# Autodesk Inventor assembly: Kopula+plus_OLED
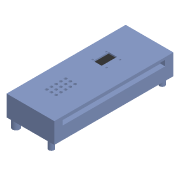
[picture p0: Inventor's stored thumbnail of the model, 180x180]
Saved by Autodesk Inventor 2021 (Build 250183000, 183)
## iProperties
Created: 2022-11-02
Part Number: Kopula+plus_OLED
Document SubType Name: Assembly
Designer: agnpi
Author: agnpi
## Documents named in this file (3)
- D:\users\agnpi\Desktop\lekcje\SEMESTR VII\INVENTOR INZ SPRAWDZONE\Kopula+plus_OLED.iam
- D:\users\agnpi\Desktop\lekcje\SEMESTR VII\INVENTOR INZ SPRAWDZONE\kopula_pod_OLED.ipt
- D:\users\agnpi\Desktop\lekcje\SEMESTR VII\INVENTOR INZ SPRAWDZONE\Pantalla OLED 0.96'' 128x64.iam
## Components (2 placed, 2 different names)
1. kopula_pod_OLED:1 — Mate:1, Mate:2, Mate:3
2. Pantalla OLED 0.96'' 128x64:1 [sub-assembly] — Mate:1, Mate:2, Mate:3
## Relationships (3: Mate 3)
- Mate:1: kopula_pod_OLED:1 ↔ Pantalla OLED 0.96'' 128x64:1
- Mate:2: kopula_pod_OLED:1 ↔ Pantalla OLED 0.96'' 128x64:1
- Mate:3: kopula_pod_OLED:1 ↔ Pantalla OLED 0.96'' 128x64:1
